# Autodesk Inventor assembly: SubAssembly Undercarriage
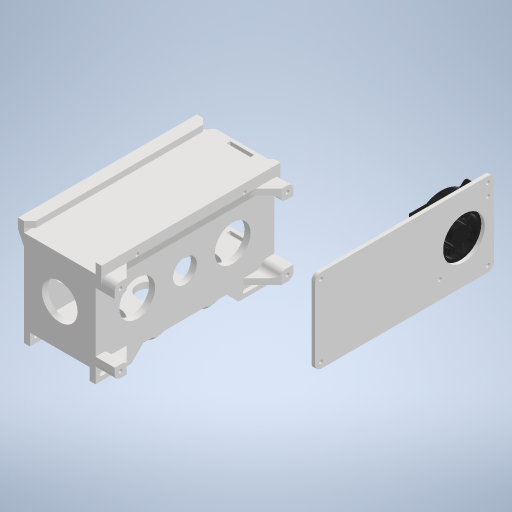
[picture p0: Inventor's stored thumbnail of the model, 512x512]
Saved by Autodesk Inventor 2023 (Build 270158000, 158)
## iProperties
Created: 2023-01-18
Part Number: SubAssembly Undercarriage
Document SubType Name: Assembly
Designer: Administrator
Author: Administrator
## Documents named in this file (4)
- C:\Users\Administrator\Documents\GitHub\WU-Team20-AutonomousDrone\CAD\ASSEMBLY\SubAssembly - Undercarriage.iam
- C:\Users\Administrator\Documents\GitHub\WU-Team20-AutonomousDrone\CAD\Electronics Mounts\BatteryCarrier SlideRail.ipt
- C:\Users\Administrator\Documents\GitHub\WU-Team20-AutonomousDrone\CAD\Raw Models\BlowerFan.ipt
- C:\Users\Administrator\Documents\GitHub\WU-Team20-AutonomousDrone\CAD\Misc\Charger ShroudPlate - EthanMockup.ipt
## Components (3 placed, 3 different names)
1. BatteryCarrier SlideRail:1
2. BlowerFan:1 — Mate:1, Mate:2
3. Charger ShroudPlate - EthanMockup:1 — Mate:1, Mate:2
## Relationships (2: Mate 2)
- Mate:1: BlowerFan:1 ↔ Charger ShroudPlate - EthanMockup:1
- Mate:2: BlowerFan:1 ↔ Charger ShroudPlate - EthanMockup:1
